# Autodesk Inventor assembly: 520 DC Gear Motor Bracket Assembly
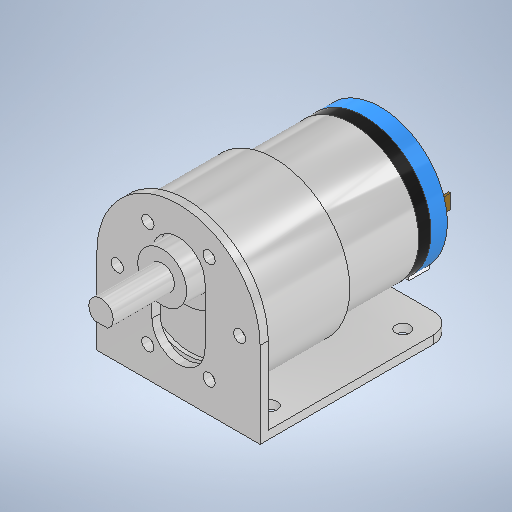
[picture p0: Inventor's stored thumbnail of the model, 512x512]
Saved by Autodesk Inventor 2025.2 (Build 292293000, 293)
## iProperties
Created: 2025-01-16
Part Number: 520 DC Gear Motor Bracket Assembly
Document SubType Name: Assembly
Designer: Matt Tidd
Author: Matt Tidd
## Documents named in this file (3)
- C:\Users\mtidd2\Desktop\H2A\CAD\Motors_and_Wheels\520 DC Gear Motor Bracket Assembly.iam
- C:\Users\mtidd2\Desktop\H2A\CAD\Motors_and_Wheels\520 DC Gear Motor Bracket.ipt
- C:\Users\mtidd2\Desktop\H2A\CAD\Motors_and_Wheels\520 DC Gear Motor.ipt
## Components (2 placed, 2 different names)
1. 520 DC Gear Motor Bracket:1 — Mate:1
2. 520 DC Gear Motor:1 — Mate:1
## Relationships (1: Mate 1)
- Mate:1: 520 DC Gear Motor Bracket:1 ↔ 520 DC Gear Motor:1
